# Autodesk Inventor assembly: Wasp Intermediate Shaft
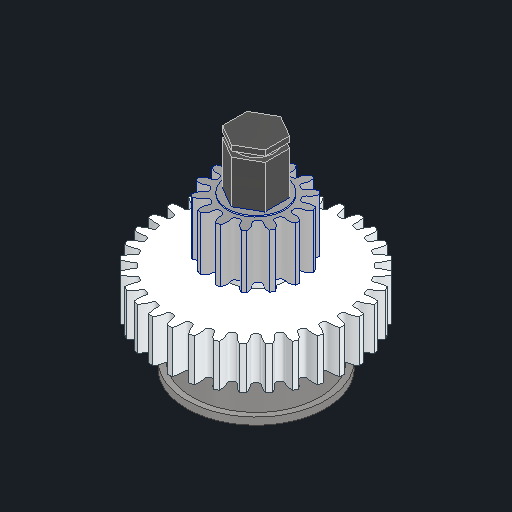
[picture p0: Inventor's stored thumbnail of the model, 512x512]
Saved by Autodesk Inventor 2022 (Build 260153000, 153)
## iProperties
Created: 2022-09-18
Part Number: Wasp Intermediate Shaft
Document SubType Name: Assembly
Designer: robpl
Author: robpl
## Documents named in this file (5)
- C:\Users\robpl\Downloads\22-20220924T142245Z-001\WASP 23-9-22\Workspaces\Workspace\Wasp Intermediate Shaft.iam
- C:\Users\robpl\Downloads\22-20220924T142245Z-001\WASP 23-9-22\Workspaces\Workspace\Wasp Intermediate Axel.ipt
- C:\Users\robpl\Downloads\22-20220924T142245Z-001\WASP 23-9-22\Workspaces\Workspace\0.375 Hex ID x 1.125 OD x 0.313 WD (Flanged Bearing) (217-2735).ipt
- C:\Users\robpl\Downloads\22-20220924T142245Z-001\WASP 23-9-22\Workspaces\Workspace\32T Aluminum Spur Gear (20 DP, 3_8_ Hex Bore) (217-5455).ipt
- C:\Users\robpl\Downloads\22-20220924T142245Z-001\WASP 23-9-22\Workspaces\Workspace\14T Aluminum Spur Gear (20 DP, 3_8_ Hex Bore) (217-2699).ipt
## Components (5 placed, 4 different names)
1. Wasp Intermediate Axel:1 — Mate:1, Mate:2, Mate:3, Mate:4, Flush:1, Mate:6, Mate:7, Mate:8, Mate:9
2. 0.375 Hex ID x 1.125 OD x 0.313 WD (Flanged Bearing) (217-2735):1 — Mate:1, Mate:2, Mate:5, Mate:10
3. 0.375 Hex ID x 1.125 OD x 0.313 WD (Flanged Bearing) (217-2735):2 — Mate:3, Mate:4, Flush:1, Mate:5
4. 32T Aluminum Spur Gear (20 DP, 3_8_ Hex Bore) (217-5455):1 — Mate:6, Mate:7, Mate:11
5. 14T Aluminum Spur Gear (20 DP, 3_8_ Hex Bore) (217-2699):1 — Mate:8, Mate:9, Mate:10, Mate:11
## Relationships (12: Mate 11, Flush 1)
- Mate:1: Wasp Intermediate Axel:1 ↔ 0.375 Hex ID x 1.125 OD x 0.313 WD (Flanged Bearing) (217-2735):1
- Mate:2: Wasp Intermediate Axel:1 ↔ 0.375 Hex ID x 1.125 OD x 0.313 WD (Flanged Bearing) (217-2735):1
- Mate:3: Wasp Intermediate Axel:1 ↔ 0.375 Hex ID x 1.125 OD x 0.313 WD (Flanged Bearing) (217-2735):2
- Mate:4: Wasp Intermediate Axel:1 ↔ 0.375 Hex ID x 1.125 OD x 0.313 WD (Flanged Bearing) (217-2735):2
- Flush:1: Wasp Intermediate Axel:1 ↔ 0.375 Hex ID x 1.125 OD x 0.313 WD (Flanged Bearing) (217-2735):2
- Mate:5 (40 mm): 0.375 Hex ID x 1.125 OD x 0.313 WD (Flanged Bearing) (217-2735):1 ↔ 0.375 Hex ID x 1.125 OD x 0.313 WD (Flanged Bearing) (217-2735):2
- Mate:6: Wasp Intermediate Axel:1 ↔ 32T Aluminum Spur Gear (20 DP, 3_8_ Hex Bore) (217-5455):1
- Mate:7: Wasp Intermediate Axel:1 ↔ 32T Aluminum Spur Gear (20 DP, 3_8_ Hex Bore) (217-5455):1
- Mate:8: Wasp Intermediate Axel:1 ↔ 14T Aluminum Spur Gear (20 DP, 3_8_ Hex Bore) (217-2699):1
- Mate:9: Wasp Intermediate Axel:1 ↔ 14T Aluminum Spur Gear (20 DP, 3_8_ Hex Bore) (217-2699):1
- Mate:10 (1 mm): 0.375 Hex ID x 1.125 OD x 0.313 WD (Flanged Bearing) (217-2735):1 ↔ 14T Aluminum Spur Gear (20 DP, 3_8_ Hex Bore) (217-2699):1
- Mate:11: 32T Aluminum Spur Gear (20 DP, 3_8_ Hex Bore) (217-5455):1 ↔ 14T Aluminum Spur Gear (20 DP, 3_8_ Hex Bore) (217-2699):1
